# Autodesk Inventor assembly: Oxxius laser subassy v2
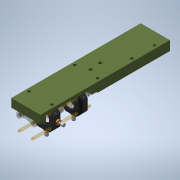
[picture p0: Inventor's stored thumbnail of the model, 180x180]
Saved by Autodesk Inventor 2022 (Build 260153000, 153)
## iProperties
Created: 2011-08-28
Part Number: Oxxius laser subassy v2
Document SubType Name: Assembly
Designer: betzige
Author: betzige
## Documents named in this file (13)
- G:\My Drive\OPM\2P-OPM_CAD\workspace\Oxxius laser subassy v2.iam
- C:\Inventor\laser combiner clone\Libraries\commercial components\Thor Labs\SM1A6 adpater SM05 internal thd to SM1 external thd\SM1A6 adpater SM05 internal thd to SM1 external thd.ipt
- G:\My Drive\OPM\2P-OPM_CAD\workspace\Imported Components\Thorlabs\SM05V05 adjustable lens tube.ipt
- G:\My Drive\OPM\2P-OPM_CAD\workspace\Imported Components\Thorlabs\CP02B cage plate adapter.ipt
- C:\Inventor\laser combiner clone\Libraries\commercial components\Thor Labs\NDM4 cage ND filter wheel\NDM4 cage ND filter wheel.ipt
- C:\Users\kk4764\Dropbox\Literature\Betzig\lattice light sheet microscope documentation\laser combiner June 2014\Workspaces\Workspace\Imported Components\CXY1 cage xy translator\CXY1 cage xy translator.ipt
- C:\Inventor\laser combiner clone\Libraries\commercial components\Oxxius\Oxxius 405 nm 250 mW LaserBoxx.ipt
- C:\Inventor\laser combiner clone\Libraries\commercial components\Thor Labs\C240TME-A mounted aspheric FL 8p0 mm NA 0p5\C240TME-A mounted aspheric FL 8p0 mm NA 0p5.ipt
- G:\My Drive\OPM\2P-OPM_CAD\workspace\Imported Components\Thorlabs\achromat 20mm FL 12p5mm dia Edmund 47-661 v2.iam
- C:\Users\kk4764\Dropbox\Literature\Betzig\lattice light sheet microscope documentation\laser combiner June 2014\Workspaces\Workspace\Imported Components\S1TM12 SM1 to M12x0p5 adapter\S1TM12 SM1 to M12x0p5 adapter.ipt
- C:\Users\kk4764\Dropbox\Literature\Betzig\lattice light sheet microscope documentation\laser combiner June 2014\Workspaces\Workspace\Oxxius laser subassy shortened baseplate.ipt
- C:\Users\kk4764\Dropbox\Literature\Betzig\lattice light sheet microscope documentation\laser combiner June 2014\Workspaces\Workspace\Imported Components\ER3 cage assy rod\ER3 cage assy rod.ipt
- C:\Users\kk4764\Dropbox\Literature\Betzig\lattice light sheet microscope documentation\laser combiner June 2014\Workspaces\Workspace\Imported Components\ER2 cage assy rod\ER2 cage assy rod.ipt
## Components (20 placed, 12 different names)
1. CXY1 cage xy translator:1 — Mate:113, Mate:114, Flush:10, Angle:11, Mate:116, Flush:20, Mate:170, Mate:184, Mate:185
2. S1TM12 SM1 to M12x0p5 adapter:2 — Mate:148, Mate:151, Mate:152, Mate:154, Flush:20
3. SM05V05 adjustable lens tube:2 — Mate:112, Mate:157, Mate:158
4. CXY1 cage xy translator:3 — Mate:110, Mate:111, Mate:114
5. SM1A6 adpater SM05 internal thd to SM1 external thd:4 — Mate:110, Mate:111, Mate:112, Mate:113
6. NDM4 cage ND filter wheel:2 — Flush:10, Angle:11, Mate:116, Mate:161, Mate:164
7. CP02B cage plate adapter:3 — Mate:159, Mate:161, Mate:170, Mate:171, Mate:172, Mate:173, Mate:182, Flush:21, Mate:183, Flush:22
8. CP02B cage plate adapter:4 — Mate:186, Mate:187, Flush:25
9. Oxxius laser subassy shortened baseplate:1 — Flush:18, Flush:19, Mate:159, Mate:171, Mate:172, Mate:173
10. Oxxius 405 nm 250 mW LaserBoxx:1 — Mate:162, Mate:163, Mate:164
11. C240TME-A mounted aspheric FL 8p0 mm NA 0p5:1 — Mate:148, Mate:150, Mate:151, Mate:155, Mate:157
12. achromat 20mm FL 12p5mm dia Edmund 47-661 v2:1 [sub-assembly] — Mate:154, Mate:155, Mate:158
13. ER3 cage assy rod:1 — Mate:174, Mate:175, Mate:185, Flush:24
14. ER3 cage assy rod:2 — Mate:176, Mate:177, Mate:184, Flush:23
15. ER3 cage assy rod:3 — Mate:178, Mate:179, Mate:183, Flush:22, Flush:23, Flush:24
16. ER3 cage assy rod:4 — Mate:180, Mate:181, Mate:182, Flush:21
17. ER2 cage assy rod:1 — Mate:174, Mate:175
18. ER2 cage assy rod:2 — Mate:176, Mate:177
19. ER2 cage assy rod:3 — Mate:178, Mate:179, Mate:186
20. ER2 cage assy rod:4 — Mate:180, Mate:181, Mate:187, Flush:25
## Relationships (48: Mate 38, Flush 9, Angle 1)
- [Mate]: CXY1 cage xy translator:1 ↔ S1TM12 SM1 to M12x0p5 adapter:2
- Mate:110: CXY1 cage xy translator:3 ↔ SM1A6 adpater SM05 internal thd to SM1 external thd:4
- Mate:111: CXY1 cage xy translator:3 ↔ SM1A6 adpater SM05 internal thd to SM1 external thd:4
- Mate:112: SM05V05 adjustable lens tube:2 ↔ SM1A6 adpater SM05 internal thd to SM1 external thd:4
- Mate:113: CXY1 cage xy translator:1 ↔ SM1A6 adpater SM05 internal thd to SM1 external thd:4
- Mate:114: CXY1 cage xy translator:1 ↔ CXY1 cage xy translator:3
- Flush:10: CXY1 cage xy translator:1 ↔ NDM4 cage ND filter wheel:2
- Angle:11 (5 deg): CXY1 cage xy translator:1 ↔ NDM4 cage ND filter wheel:2
- Mate:116: CXY1 cage xy translator:1 ↔ NDM4 cage ND filter wheel:2
- Flush:18: Oxxius laser subassy shortened baseplate:1
- Flush:19 (-40 mm): Oxxius laser subassy shortened baseplate:1
- Mate:148: S1TM12 SM1 to M12x0p5 adapter:2 ↔ C240TME-A mounted aspheric FL 8p0 mm NA 0p5:1
- Mate:150: C240TME-A mounted aspheric FL 8p0 mm NA 0p5:1
- Mate:151: S1TM12 SM1 to M12x0p5 adapter:2 ↔ C240TME-A mounted aspheric FL 8p0 mm NA 0p5:1
- Mate:152: S1TM12 SM1 to M12x0p5 adapter:2
- Mate:154: S1TM12 SM1 to M12x0p5 adapter:2 ↔ achromat 20mm FL 12p5mm dia Edmund 47-661 v2:1
- Mate:155: C240TME-A mounted aspheric FL 8p0 mm NA 0p5:1 ↔ achromat 20mm FL 12p5mm dia Edmund 47-661 v2:1
- Mate:157: SM05V05 adjustable lens tube:2 ↔ C240TME-A mounted aspheric FL 8p0 mm NA 0p5:1
- Mate:158: SM05V05 adjustable lens tube:2 ↔ achromat 20mm FL 12p5mm dia Edmund 47-661 v2:1
- Mate:159: CP02B cage plate adapter:3 ↔ Oxxius laser subassy shortened baseplate:1
- Mate:161 (-25 mm): NDM4 cage ND filter wheel:2 ↔ CP02B cage plate adapter:3
- Flush:20: CXY1 cage xy translator:1 ↔ S1TM12 SM1 to M12x0p5 adapter:2
- Mate:162: Oxxius 405 nm 250 mW LaserBoxx:1
- Mate:163: Oxxius 405 nm 250 mW LaserBoxx:1
- Mate:164 (15 mm): NDM4 cage ND filter wheel:2 ↔ Oxxius 405 nm 250 mW LaserBoxx:1
- Mate:170: CXY1 cage xy translator:1 ↔ CP02B cage plate adapter:3
- Mate:171: CP02B cage plate adapter:3 ↔ Oxxius laser subassy shortened baseplate:1
- Mate:172: CP02B cage plate adapter:3 ↔ Oxxius laser subassy shortened baseplate:1
- Mate:173: CP02B cage plate adapter:3 ↔ Oxxius laser subassy shortened baseplate:1
- Mate:174: ER3 cage assy rod:1 ↔ ER2 cage assy rod:1
- Mate:175: ER3 cage assy rod:1 ↔ ER2 cage assy rod:1
- Mate:176: ER3 cage assy rod:2 ↔ ER2 cage assy rod:2
- Mate:177: ER3 cage assy rod:2 ↔ ER2 cage assy rod:2
- Mate:178: ER3 cage assy rod:3 ↔ ER2 cage assy rod:3
- Mate:179: ER3 cage assy rod:3 ↔ ER2 cage assy rod:3
- Mate:180: ER3 cage assy rod:4 ↔ ER2 cage assy rod:4
- Mate:181: ER3 cage assy rod:4 ↔ ER2 cage assy rod:4
- Mate:182: CP02B cage plate adapter:3 ↔ ER3 cage assy rod:4
- Flush:21: CP02B cage plate adapter:3 ↔ ER3 cage assy rod:4
- Mate:183: CP02B cage plate adapter:3 ↔ ER3 cage assy rod:3
- Flush:22: CP02B cage plate adapter:3 ↔ ER3 cage assy rod:3
- Mate:184: CXY1 cage xy translator:1 ↔ ER3 cage assy rod:2
- Flush:23: ER3 cage assy rod:2 ↔ ER3 cage assy rod:3
- Mate:185: CXY1 cage xy translator:1 ↔ ER3 cage assy rod:1
- Flush:24: ER3 cage assy rod:1 ↔ ER3 cage assy rod:3
- Mate:186: CP02B cage plate adapter:4 ↔ ER2 cage assy rod:3
- Mate:187: CP02B cage plate adapter:4 ↔ ER2 cage assy rod:4
- Flush:25: CP02B cage plate adapter:4 ↔ ER2 cage assy rod:4
